# Autodesk Inventor assembly: jamming_gripper
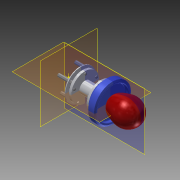
[picture p0: Inventor's stored thumbnail of the model, 180x180]
Saved by Autodesk Inventor 2015 (Build 190159000, 159)
## iProperties
Created: 2015-12-22
Part Number: jamming_gripper
Document SubType Name: Assembly
Designer: Ryo
Author: Ryo
## Documents named in this file (11)
- D:\Users\Ryo\Documents\Inventor\motoman_cad\SIA5_TOOL\jamming_gripper.iam
- D:\Users\Ryo\Documents\Inventor\motoman_cad\SIA5_TOOL\tool_1.ipt
- D:\Users\Ryo\Documents\Inventor\motoman_cad\SIA5_TOOL\tool_2_MIR.ipt
- D:\Users\Ryo\Documents\Inventor\Content Center Files\R2015\ja-JP\JIS B 1256(3)\JIS B 1256 - 4.8(3).ipt
- D:\Users\Ryo\Documents\Inventor\Content Center Files\R2015\ja-JP\JIS B 1176\JIS B 1176 - M4 x 12.ipt
- D:\Users\Ryo\Documents\Inventor\motoman_cad\SIA5_TOOL\tool_3.ipt
- D:\Users\Ryo\Documents\Inventor\motoman_cad\SIA5_TOOL\plate.ipt
- D:\Users\Ryo\Documents\Inventor\motoman_cad\SIA5_TOOL\pillar.ipt
- D:\Users\Ryo\Documents\Inventor\Content Center Files\R2015\ja-JP\JIS B 1176\JIS B 1176 - M5 x 30.ipt
- D:\Users\Ryo\Documents\Inventor\Content Center Files\R2015\ja-JP\JIS B 1176\JIS B 1176 - M3 x 16.ipt
- D:\Users\Ryo\Documents\Inventor\Content Center Files\R2015\ja-JP\JIS B 1181  A B\JIS B 1181 - A_B M3.5.ipt
## Components (31 placed, 10 different names)
1. tool_1:1 — メイト:1, メイト:2, メイト:3, メイト:4, メイト:5, メイト:6, メイト:7, メイト:8, メイト:9, メイト:10, メイト:11, メイト:12, メイト:13, 挿入:2, メイト:14, メイト:25, メイト:26, メイト:27, 挿入:14, 挿入:15, 挿入:16, 挿入:17, メイト:29
2. tool_2_MIR:1 — メイト:1, メイト:2, メイト:3, メイト:16, 正接:1
3. JIS B 1256 4.8:1 — メイト:4, メイト:5, 挿入:4
4. JIS B 1256 4.8:2 — メイト:6, メイト:7, 挿入:1
5. JIS B 1256 4.8:3 — メイト:8, メイト:9, メイト:15
6. JIS B 1256 4.8:4 — メイト:10, メイト:11, 挿入:3
7. JIS B 1256 4.8:5 — メイト:12, メイト:13
8. JIS B 1176 - メートル M4 x 12:1 — 挿入:1
9. JIS B 1176 - メートル M4 x 12:2 — 挿入:2
10. JIS B 1176 - メートル M4 x 12:3 — 挿入:3
11. JIS B 1176 - メートル M4 x 12:4 — メイト:14, メイト:15
12. JIS B 1176 - メートル M4 x 12:5 — 挿入:4
13. tool_3:1 — メイト:16, 正接:1
14. plate:1 — メイト:17, メイト:18, メイト:19, メイト:20, メイト:21, メイト:22, メイト:23, メイト:24, 挿入:6, 挿入:7, 挿入:8, 挿入:9, メイト:25, メイト:26, 挿入:10, 挿入:11, 挿入:12, 挿入:13
15. pillar:1 — メイト:23, メイト:24, 挿入:5
16. pillar:2 — メイト:21, メイト:22
17. pillar:3 — メイト:19, メイト:20, メイト:28
18. pillar:4 — メイト:17, メイト:18
19. JIS B 1176 - メートル M5 x 30:1 — 挿入:5
20. JIS B 1176 - メートル M5 x 30:2 — 挿入:6
21. JIS B 1176 - メートル M5 x 30:3 — 挿入:7, メイト:27
22. JIS B 1176 - メートル M5 x 30:4 — 挿入:8
23. JIS B 1176 - メートル M5 x 30:5 — 挿入:9
24. JIS B 1176 - メートル M3 x 16:1 — 挿入:10
25. JIS B 1176 - メートル M3 x 16:2 — 挿入:11
26. JIS B 1176 - メートル M3 x 16:3 — 挿入:12
27. JIS B 1176 - メートル M3 x 16:4 — 挿入:13
28. JIS B 1181 A/B - メートル A/B M3.5:1 — 挿入:14
29. JIS B 1181 A/B - メートル A/B M3.5:2 — 挿入:15
30. JIS B 1181 A/B - メートル A/B M3.5:3 — 挿入:16
31. JIS B 1181 A/B - メートル A/B M3.5:4 — 挿入:17
## Relationships (47: Mate 29, Insert 17, Tangent 1)
- メイト:1 [Mate]: tool_1:1 ↔ tool_2_MIR:1
- メイト:2 [Mate]: tool_1:1 ↔ tool_2_MIR:1
- メイト:3 [Mate]: tool_1:1 ↔ tool_2_MIR:1
- メイト:4 [Mate]: tool_1:1 ↔ JIS B 1256 4.8:1
- メイト:5 [Mate]: tool_1:1 ↔ JIS B 1256 4.8:1
- メイト:6 [Mate]: tool_1:1 ↔ JIS B 1256 4.8:2
- メイト:7 [Mate]: tool_1:1 ↔ JIS B 1256 4.8:2
- メイト:8 [Mate]: tool_1:1 ↔ JIS B 1256 4.8:3
- メイト:9 [Mate]: tool_1:1 ↔ JIS B 1256 4.8:3
- メイト:10 [Mate]: tool_1:1 ↔ JIS B 1256 4.8:4
- メイト:11 [Mate]: tool_1:1 ↔ JIS B 1256 4.8:4
- メイト:12 [Mate]: tool_1:1 ↔ JIS B 1256 4.8:5
- メイト:13 [Mate]: tool_1:1 ↔ JIS B 1256 4.8:5
- 挿入:1 [Insert]: JIS B 1256 4.8:2 ↔ JIS B 1176 - メートル M4 x 12:1
- 挿入:2 [Insert]: tool_1:1 ↔ JIS B 1176 - メートル M4 x 12:2
- 挿入:3 [Insert]: JIS B 1256 4.8:4 ↔ JIS B 1176 - メートル M4 x 12:3
- メイト:14 [Mate]: tool_1:1 ↔ JIS B 1176 - メートル M4 x 12:4
- メイト:15 [Mate]: JIS B 1256 4.8:3 ↔ JIS B 1176 - メートル M4 x 12:4
- 挿入:4 [Insert]: JIS B 1256 4.8:1 ↔ JIS B 1176 - メートル M4 x 12:5
- メイト:16 [Mate]: tool_2_MIR:1 ↔ tool_3:1
- 正接:1 [Tangent]: tool_2_MIR:1 ↔ tool_3:1
- メイト:17 [Mate]: plate:1 ↔ pillar:4
- メイト:18 [Mate]: plate:1 ↔ pillar:4
- メイト:19 [Mate]: plate:1 ↔ pillar:3
- メイト:20 [Mate]: plate:1 ↔ pillar:3
- メイト:21 [Mate]: plate:1 ↔ pillar:2
- メイト:22 [Mate]: plate:1 ↔ pillar:2
- メイト:23 [Mate]: plate:1 ↔ pillar:1
- メイト:24 [Mate]: plate:1 ↔ pillar:1
- 挿入:5 [Insert]: pillar:1 ↔ JIS B 1176 - メートル M5 x 30:1
- 挿入:6 [Insert]: plate:1 ↔ JIS B 1176 - メートル M5 x 30:2
- 挿入:7 [Insert]: plate:1 ↔ JIS B 1176 - メートル M5 x 30:3
- 挿入:8 [Insert]: plate:1 ↔ JIS B 1176 - メートル M5 x 30:4
- 挿入:9 [Insert]: plate:1 ↔ JIS B 1176 - メートル M5 x 30:5
- メイト:25 [Mate]: tool_1:1 ↔ plate:1
- メイト:26 [Mate]: tool_1:1 ↔ plate:1
- メイト:27 [Mate]: tool_1:1 ↔ JIS B 1176 - メートル M5 x 30:3
- 挿入:10 [Insert]: plate:1 ↔ JIS B 1176 - メートル M3 x 16:1
- 挿入:11 [Insert]: plate:1 ↔ JIS B 1176 - メートル M3 x 16:2
- 挿入:12 [Insert]: plate:1 ↔ JIS B 1176 - メートル M3 x 16:3
- 挿入:13 [Insert]: plate:1 ↔ JIS B 1176 - メートル M3 x 16:4
- 挿入:14 [Insert]: tool_1:1 ↔ JIS B 1181 A/B - メートル A/B M3.5:1
- 挿入:15 [Insert]: tool_1:1 ↔ JIS B 1181 A/B - メートル A/B M3.5:2
- 挿入:16 [Insert]: tool_1:1 ↔ JIS B 1181 A/B - メートル A/B M3.5:3
- 挿入:17 [Insert]: tool_1:1 ↔ JIS B 1181 A/B - メートル A/B M3.5:4
- メイト:28 [Mate]: pillar:3
- メイト:29 [Mate]: tool_1:1
